# Autodesk Inventor assembly: leg_upper_right
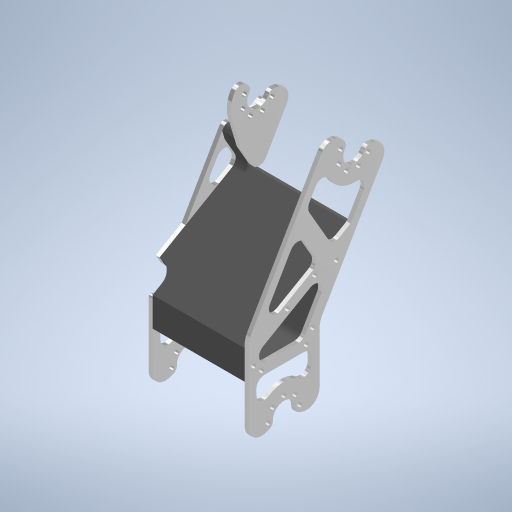
[picture p0: Inventor's stored thumbnail of the model, 512x512]
Saved by Autodesk Inventor 2024.1 (Build 281209000, 209)
## iProperties
Created: 2024-10-11
Part Number: leg_upper_right
Document SubType Name: Assembly
Designer: hibik
Author: hibik
## Documents named in this file (6)
- C:\Users\hibik\Documents\Robomech\HR\Eglantyne\hard\leg\leg_upper_right.iam
- C:\Users\hibik\Documents\Robomech\HR\Eglantyne\hard\leg\leg_upper_outside.ipt
- C:\Users\hibik\Documents\Robomech\HR\Eglantyne\hard\leg\leg_upper_middle_right.ipt
- C:\Users\hibik\Documents\Robomech\HR\Eglantyne\hard\leg\leg_upper_inside_down.ipt
- C:\Users\hibik\Documents\Robomech\HR\Eglantyne\hard\leg\leg_upper_inside_up_base.ipt
- C:\Users\hibik\Documents\Robomech\HR\Eglantyne\hard\leg\leg_upper_inside_up.ipt
## Components (5 placed, 5 different names)
1. leg_upper_outside:1 — フラッシュ:1, フラッシュ:2, メイト:1, 挿入:1, フラッシュ:3
2. leg_upper_middle_right:1 — 挿入:1, フラッシュ:3, 挿入:2, 挿入:3, フラッシュ:4, メイト:2, フラッシュ:5, フラッシュ:6, フラッシュ:8
3. leg_upper_inside_down:1 — 挿入:2, 挿入:3, フラッシュ:7
4. leg_upper_inside_up:1 — フラッシュ:4, メイト:2, フラッシュ:5
5. leg_upper_inside_up_base:1 — フラッシュ:6, フラッシュ:7, フラッシュ:8
## Relationships (13: Flush 8, Insert 3, Mate 2)
- フラッシュ:1 [Flush]: leg_upper_outside:1
- フラッシュ:2 [Flush]: leg_upper_outside:1
- メイト:1 [Mate]: leg_upper_outside:1
- 挿入:1 [Insert]: leg_upper_outside:1 ↔ leg_upper_middle_right:1
- フラッシュ:3 [Flush]: leg_upper_outside:1 ↔ leg_upper_middle_right:1
- 挿入:2 [Insert]: leg_upper_middle_right:1 ↔ leg_upper_inside_down:1
- 挿入:3 [Insert]: leg_upper_middle_right:1 ↔ leg_upper_inside_down:1
- フラッシュ:4 [Flush]: leg_upper_middle_right:1 ↔ leg_upper_inside_up:1
- メイト:2 [Mate]: leg_upper_middle_right:1 ↔ leg_upper_inside_up:1
- フラッシュ:5 [Flush]: leg_upper_middle_right:1 ↔ leg_upper_inside_up:1
- フラッシュ:6 [Flush]: leg_upper_middle_right:1 ↔ leg_upper_inside_up_base:1
- フラッシュ:7 [Flush]: leg_upper_inside_down:1 ↔ leg_upper_inside_up_base:1
- フラッシュ:8 [Flush]: leg_upper_middle_right:1 ↔ leg_upper_inside_up_base:1
